# Autodesk Inventor assembly: 000 Ensamblaje 3d_LM-Cable_Forming - TOP00
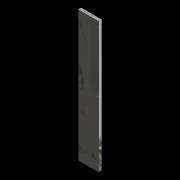
[picture p0: Inventor's stored thumbnail of the model, 180x180]
Saved by Autodesk Inventor 2018.3 (Build 223284000, 284)
## iProperties
Category: 0
Created: 2026-02-11
Part Number: 000 Ensamblaje 3d_LM-Cable_Forming - TOP00
Document SubType Name: Assembly
Designer: aca6
Manufacturer-1: {"Link": "", "Name": "Embention Sistemas Inteligentes S.A.", "PartNumber": "3d_LM-Cable_Forming - TOP00", "partner_id": false}
Manufacturer-2: {"Link": "", "Name": "", "PartNumber": "", "partner_id": false}
Manufacturer-3: {"Link": "", "Name": "", "PartNumber": "", "partner_id": false}
Manufacturer-4: {"Link": "", "Name": "", "PartNumber": "", "partner_id": false}
Manufacturer-5: {"Link": "", "Name": "", "PartNumber": "", "partner_id": false}
Provider-1: {"Link": "", "Name": "", "PartNumber": "", "partner_id": false}
Provider-2: {"Link": "", "Name": "", "PartNumber": "", "partner_id": false}
Provider-3: {"Link": "", "Name": "", "PartNumber": "", "partner_id": false}
Provider-4: {"Link": "", "Name": "", "PartNumber": "", "partner_id": false}
Provider-5: {"Link": "", "Name": "", "PartNumber": "", "partner_id": false}
odoo_id: 19248
odoo_item_code: 3d_LM-Cable_Forming
odoo_internal_code: False
odoo_pt_internal_code: PT12083
odoo_part_number_code: False
odoo_model: product.template
odoo_x2o_application_version: 12.0.4.20
odoo_d2o_version: 12.0.1.6.0
Author: aca6
## Documents named in this file (4)
- C:\Users\aca6\git\LM\items\3d_LM\items\LM-Cable_Forming\items\3d_LM-Cable_Forming\variants\TOP00\3d\000 Ensamblaje 3d_LM-Cable_Forming - TOP00.iam
- C:\Users\aca6\git\LM\items\3d_LM\items\LM-Cable_Forming\items\3d_LM-Cable_Forming\variants\TOP00\3d\3d_LM-Cable_Forming - Top mold.ipt
- C:\Users\aca6\git\LM\items\3d_LM\3d\3d_LM - Top Wire - Phantom.ipt
- C:\Users\aca6\git\LM\items\_accesories\Pasadores\3d_Fabory\3d\DIN 7\DIN 7 4x8 mm Inox A4.ipt
## Components (9 placed, 3 different names)
1. 3d_LM-Cable_Forming - Top mold:1 — Mate:1, Flush:1, Flush:2, Flush:3, Mate:4, Mate:5, Mate:6, Mate:7, Mate:8, Mate:9
2. 3d_LM-Cable_Forming - Top mold:2 — Mate:1, Flush:1, Flush:2, Mate:2, Mate:3, Flush:4, Flush:5, Flush:6, Flush:7, Flush:8, Flush:9
3. 3d_LM - Top Wire - Phantom:1 — Mate:2, Mate:3, Flush:3
4. DIN 7 4x8 mm Inox A4:1 — Mate:4, Flush:4
5. DIN 7 4x8 mm Inox A4:2 — Mate:5, Flush:5
6. DIN 7 4x8 mm Inox A4:3 — Mate:6, Flush:7
7. DIN 7 4x8 mm Inox A4:4 — Mate:7, Flush:6
8. DIN 7 4x8 mm Inox A4:5 — Mate:8, Flush:8
9. DIN 7 4x8 mm Inox A4:6 — Mate:9, Flush:9
## Relationships (18: Mate 9, Flush 9)
- Mate:1: 3d_LM-Cable_Forming - Top mold:1 ↔ 3d_LM-Cable_Forming - Top mold:2
- Flush:1: 3d_LM-Cable_Forming - Top mold:1 ↔ 3d_LM-Cable_Forming - Top mold:2
- Flush:2: 3d_LM-Cable_Forming - Top mold:1 ↔ 3d_LM-Cable_Forming - Top mold:2
- Mate:2: 3d_LM-Cable_Forming - Top mold:2 ↔ 3d_LM - Top Wire - Phantom:1
- Mate:3: 3d_LM-Cable_Forming - Top mold:2 ↔ 3d_LM - Top Wire - Phantom:1
- Flush:3: 3d_LM-Cable_Forming - Top mold:1 ↔ 3d_LM - Top Wire - Phantom:1
- Mate:4: 3d_LM-Cable_Forming - Top mold:1 ↔ DIN 7 4x8 mm Inox A4:1
- Mate:5: 3d_LM-Cable_Forming - Top mold:1 ↔ DIN 7 4x8 mm Inox A4:2
- Mate:6: 3d_LM-Cable_Forming - Top mold:1 ↔ DIN 7 4x8 mm Inox A4:3
- Mate:7: 3d_LM-Cable_Forming - Top mold:1 ↔ DIN 7 4x8 mm Inox A4:4
- Mate:8: 3d_LM-Cable_Forming - Top mold:1 ↔ DIN 7 4x8 mm Inox A4:5
- Mate:9: 3d_LM-Cable_Forming - Top mold:1 ↔ DIN 7 4x8 mm Inox A4:6
- Flush:4: 3d_LM-Cable_Forming - Top mold:2 ↔ DIN 7 4x8 mm Inox A4:1
- Flush:5: 3d_LM-Cable_Forming - Top mold:2 ↔ DIN 7 4x8 mm Inox A4:2
- Flush:6: 3d_LM-Cable_Forming - Top mold:2 ↔ DIN 7 4x8 mm Inox A4:4
- Flush:7: 3d_LM-Cable_Forming - Top mold:2 ↔ DIN 7 4x8 mm Inox A4:3
- Flush:8: 3d_LM-Cable_Forming - Top mold:2 ↔ DIN 7 4x8 mm Inox A4:5
- Flush:9: 3d_LM-Cable_Forming - Top mold:2 ↔ DIN 7 4x8 mm Inox A4:6
